# Autodesk Inventor assembly: Y_rail_Assembly_Rev3
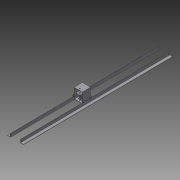
[picture p0: Inventor's stored thumbnail of the model, 180x180]
Saved by Autodesk Inventor 2015 (Build 190159000, 159)
## iProperties
Created: 2017-01-11
Part Number: Y_rail_Assembly_Rev3
Document SubType Name: Assembly
Designer: Guy
Mass: 1796.89 g
Surface Area: 4829.55 cm^2
Volume: 1200.62 cm^3
Density: 1.49664 g/cm^3
Author: Guy
## Documents named in this file (10)
- C:\Users\Guy\Documents\Fourth Year\Capstone\git\Capstone-Project\doc\CAD\LowLevel_Rev3\Y_rail_Assembly_Rev3.iam
- C:\Users\Guy\Documents\Fourth Year\Capstone\git\Capstone-Project\doc\CAD\LowLevel_Rev3\Y_Rail-SquareBar-Rev3.ipt
- C:\Users\Guy\Documents\Fourth Year\Capstone\git\Capstone-Project\doc\CAD\LowLevel_Rev3\XY_Wheel-SquareBar-Rev3.ipt
- C:\Users\Guy\Documents\Fourth Year\Capstone\git\Capstone-Project\doc\CAD\LowLevel_Rev3\EE_Base-SquareBar-Rev3.ipt
- C:\Users\Guy\Documents\Fourth Year\Capstone\git\Capstone-Project\doc\CAD\LowLevel_Rev3\Y_rail_Assembly_Rev3\Design Accelerator\Spur Gears1.iam
- C:\Users\Guy\Documents\Fourth Year\Capstone\git\Capstone-Project\doc\CAD\LowLevel_Rev3\Stepper_Motor_Holder-SquareBar-Rev3.ipt
- C:\Users\Guy\Documents\Fourth Year\Capstone\git\Capstone-Project\doc\CAD\Stepper Motor\NEMA 17-old\M1173041- NEMA 17.ipt
- C:\Users\Guy\Documents\Fourth Year\Capstone\git\Capstone-Project\doc\CAD\Nuts and Bolts\3-16in_1 1-4in_Bolt.ipt
- C:\Users\Guy\Documents\Fourth Year\Capstone\git\Capstone-Project\doc\CAD\Nuts and Bolts\3-16in_7-16in_washer(num8).ipt
- C:\Users\Guy\Documents\Fourth Year\Capstone\git\Capstone-Project\doc\CAD\Nuts and Bolts\3-16in_1-16in_nut(num2).ipt
## Components (34 placed, 9 different names)
1. Y_Rail-SquareBar-Rev3:1 — Tangent:1, Tangent:2, Mate:39, Mate:97, Mate:99
2. Y_Rail-SquareBar-Rev3:2 — Tangent:3, Tangent:4, Mate:12, Mate:97, Mate:99
3. XY_Wheel-SquareBar-Rev3:1 — Tangent:1, Mate:9, Flush:2, Mate:39, Mate:45, Mate:51
4. XY_Wheel-SquareBar-Rev3:2 — Tangent:4, Mate:9, Flush:4, Mate:15, Mate:71, Mate:84, Mate:92, Mate:95
5. XY_Wheel-SquareBar-Rev3:3 — Tangent:3, Mate:10, Mate:12, Flush:4, Mate:14, Mate:54, Mate:64, Mate:65
6. XY_Wheel-SquareBar-Rev3:4 — Tangent:2, Mate:10, Flush:2, Mate:13, Mate:73, Mate:79, Mate:80
7. Spur Gears:1 [sub-assembly] — Mate:17, Mate:36, Flush:5
8. EE_Base-SquareBar-Rev3:1 — Mate:13, Mate:14, Mate:15, Mate:17, Mate:37, Mate:38, Mate:53, Mate:55, Mate:63, Mate:68, Mate:69, Mate:71, Mate:72, Mate:74, Mate:85, Mate:88, Mate:98, Mate:100, Mate:101
9. M1173041- NEMA 17:1 — Mate:36, Flush:5, Mate:69, Mate:70, Mate:98
10. 3-16in_1 1-4in_Bolt:1 — Mate:37, Mate:38, Mate:44, Mate:46, Mate:48, Mate:49, Mate:52
11. 3-16in_7-16in_washer(num8):3 — Mate:44, Mate:45, Mate:47
12. 3-16in_1-16in_nut(num2):1 — Mate:46, Mate:47
13. 3-16in_7-16in_washer(num8):4 — Mate:48, Mate:50, Mate:51
14. 3-16in_1-16in_nut(num2):2 — Mate:49, Mate:50
15. 3-16in_1-16in_nut(num2):3 — Mate:52, Mate:53
16. 3-16in_1 1-4in_Bolt:2 — Mate:54, Mate:55, Mate:56, Mate:57, Mate:58, Mate:59, Mate:60
17. 3-16in_1-16in_nut(num2):4 — Mate:56, Mate:61
18. 3-16in_1-16in_nut(num2):5 — Mate:58, Mate:63
19. 3-16in_1-16in_nut(num2):6 — Mate:59, Mate:62
20. 3-16in_7-16in_washer(num8):5 — Mate:57, Mate:62, Mate:64
21. 3-16in_7-16in_washer(num8):6 — Mate:60, Mate:61, Mate:65
22. Stepper_Motor_Holder-SquareBar-Rev3:1 — Mate:68, Mate:70, Mate:100, Mate:101
23. 3-16in_1 1-4in_Bolt:3 — Mate:84, Mate:85, Mate:89, Mate:90, Mate:91, Mate:93, Mate:94
24. 3-16in_1 1-4in_Bolt:4 — Mate:72, Mate:73, Mate:75, Mate:77, Mate:78, Mate:82, Mate:83
25. 3-16in_1-16in_nut(num2):7 — Mate:86, Mate:91
26. 3-16in_1-16in_nut(num2):8 — Mate:87, Mate:94
27. 3-16in_1-16in_nut(num2):9 — Mate:88, Mate:89
28. 3-16in_1-16in_nut(num2):10 — Mate:76, Mate:78
29. 3-16in_1-16in_nut(num2):11 — Mate:81, Mate:82
30. 3-16in_1-16in_nut(num2):12 — Mate:74, Mate:75
31. 3-16in_7-16in_washer(num8):7 — Mate:80, Mate:81, Mate:83
32. 3-16in_7-16in_washer(num8):8 — Mate:87, Mate:93, Mate:95
33. 3-16in_7-16in_washer(num8):9 — Mate:76, Mate:77, Mate:79
34. 3-16in_7-16in_washer(num8):10 — Mate:86, Mate:90, Mate:92
## Relationships (73: Mate 66, Tangent 4, Flush 3)
- Tangent:1: Y_Rail-SquareBar-Rev3:1 ↔ XY_Wheel-SquareBar-Rev3:1
- Tangent:2: Y_Rail-SquareBar-Rev3:1 ↔ XY_Wheel-SquareBar-Rev3:4
- Tangent:3: Y_Rail-SquareBar-Rev3:2 ↔ XY_Wheel-SquareBar-Rev3:3
- Tangent:4: Y_Rail-SquareBar-Rev3:2 ↔ XY_Wheel-SquareBar-Rev3:2
- Mate:9: XY_Wheel-SquareBar-Rev3:1 ↔ XY_Wheel-SquareBar-Rev3:2
- Mate:10: XY_Wheel-SquareBar-Rev3:3 ↔ XY_Wheel-SquareBar-Rev3:4
- Flush:2: XY_Wheel-SquareBar-Rev3:1 ↔ XY_Wheel-SquareBar-Rev3:4
- Mate:12 (1.75 mm): Y_Rail-SquareBar-Rev3:2 ↔ XY_Wheel-SquareBar-Rev3:3
- Flush:4: XY_Wheel-SquareBar-Rev3:2 ↔ XY_Wheel-SquareBar-Rev3:3
- Mate:13: XY_Wheel-SquareBar-Rev3:4 ↔ EE_Base-SquareBar-Rev3:1
- Mate:14: XY_Wheel-SquareBar-Rev3:3 ↔ EE_Base-SquareBar-Rev3:1
- Mate:15: XY_Wheel-SquareBar-Rev3:2 ↔ EE_Base-SquareBar-Rev3:1
- Mate:17: Spur Gears:1 ↔ EE_Base-SquareBar-Rev3:1
- Mate:36: Spur Gears:1 ↔ M1173041- NEMA 17:1
- Flush:5 (-10 mm): Spur Gears:1 ↔ M1173041- NEMA 17:1
- Mate:37: EE_Base-SquareBar-Rev3:1 ↔ 3-16in_1 1-4in_Bolt:1
- Mate:38: EE_Base-SquareBar-Rev3:1 ↔ 3-16in_1 1-4in_Bolt:1
- Mate:39: Y_Rail-SquareBar-Rev3:1 ↔ XY_Wheel-SquareBar-Rev3:1
- Mate:44: 3-16in_1 1-4in_Bolt:1 ↔ 3-16in_7-16in_washer(num8):3
- Mate:45: XY_Wheel-SquareBar-Rev3:1 ↔ 3-16in_7-16in_washer(num8):3
- Mate:46: 3-16in_1 1-4in_Bolt:1 ↔ 3-16in_1-16in_nut(num2):1
- Mate:47: 3-16in_7-16in_washer(num8):3 ↔ 3-16in_1-16in_nut(num2):1
- Mate:48: 3-16in_1 1-4in_Bolt:1 ↔ 3-16in_7-16in_washer(num8):4
- Mate:49: 3-16in_1 1-4in_Bolt:1 ↔ 3-16in_1-16in_nut(num2):2
- Mate:50: 3-16in_7-16in_washer(num8):4 ↔ 3-16in_1-16in_nut(num2):2
- Mate:51: XY_Wheel-SquareBar-Rev3:1 ↔ 3-16in_7-16in_washer(num8):4
- Mate:52: 3-16in_1 1-4in_Bolt:1 ↔ 3-16in_1-16in_nut(num2):3
- Mate:53: EE_Base-SquareBar-Rev3:1 ↔ 3-16in_1-16in_nut(num2):3
- Mate:54: XY_Wheel-SquareBar-Rev3:3 ↔ 3-16in_1 1-4in_Bolt:2
- Mate:55: EE_Base-SquareBar-Rev3:1 ↔ 3-16in_1 1-4in_Bolt:2
- Mate:56: 3-16in_1 1-4in_Bolt:2 ↔ 3-16in_1-16in_nut(num2):4
- Mate:57: 3-16in_1 1-4in_Bolt:2 ↔ 3-16in_7-16in_washer(num8):5
- Mate:58: 3-16in_1 1-4in_Bolt:2 ↔ 3-16in_1-16in_nut(num2):5
- Mate:59: 3-16in_1 1-4in_Bolt:2 ↔ 3-16in_1-16in_nut(num2):6
- Mate:60: 3-16in_1 1-4in_Bolt:2 ↔ 3-16in_7-16in_washer(num8):6
- Mate:61: 3-16in_1-16in_nut(num2):4 ↔ 3-16in_7-16in_washer(num8):6
- Mate:62: 3-16in_1-16in_nut(num2):6 ↔ 3-16in_7-16in_washer(num8):5
- Mate:63: EE_Base-SquareBar-Rev3:1 ↔ 3-16in_1-16in_nut(num2):5
- Mate:64: XY_Wheel-SquareBar-Rev3:3 ↔ 3-16in_7-16in_washer(num8):5
- Mate:65: XY_Wheel-SquareBar-Rev3:3 ↔ 3-16in_7-16in_washer(num8):6
- Mate:68: EE_Base-SquareBar-Rev3:1 ↔ Stepper_Motor_Holder-SquareBar-Rev3:1
- Mate:69: EE_Base-SquareBar-Rev3:1 ↔ M1173041- NEMA 17:1
- Mate:70: M1173041- NEMA 17:1 ↔ Stepper_Motor_Holder-SquareBar-Rev3:1
- Mate:71 (5.625 mm): XY_Wheel-SquareBar-Rev3:2 ↔ EE_Base-SquareBar-Rev3:1
- Mate:72: EE_Base-SquareBar-Rev3:1 ↔ 3-16in_1 1-4in_Bolt:4
- Mate:73: XY_Wheel-SquareBar-Rev3:4 ↔ 3-16in_1 1-4in_Bolt:4
- Mate:74: EE_Base-SquareBar-Rev3:1 ↔ 3-16in_1-16in_nut(num2):12
- Mate:75: 3-16in_1 1-4in_Bolt:4 ↔ 3-16in_1-16in_nut(num2):12
- Mate:76: 3-16in_1-16in_nut(num2):10 ↔ 3-16in_7-16in_washer(num8):9
- Mate:77: 3-16in_1 1-4in_Bolt:4 ↔ 3-16in_7-16in_washer(num8):9
- Mate:78: 3-16in_1 1-4in_Bolt:4 ↔ 3-16in_1-16in_nut(num2):10
- Mate:79: XY_Wheel-SquareBar-Rev3:4 ↔ 3-16in_7-16in_washer(num8):9
- Mate:80: XY_Wheel-SquareBar-Rev3:4 ↔ 3-16in_7-16in_washer(num8):7
- Mate:81: 3-16in_1-16in_nut(num2):11 ↔ 3-16in_7-16in_washer(num8):7
- Mate:82: 3-16in_1 1-4in_Bolt:4 ↔ 3-16in_1-16in_nut(num2):11
- Mate:83: 3-16in_1 1-4in_Bolt:4 ↔ 3-16in_7-16in_washer(num8):7
- Mate:84: XY_Wheel-SquareBar-Rev3:2 ↔ 3-16in_1 1-4in_Bolt:3
- Mate:85: EE_Base-SquareBar-Rev3:1 ↔ 3-16in_1 1-4in_Bolt:3
- Mate:86: 3-16in_1-16in_nut(num2):7 ↔ 3-16in_7-16in_washer(num8):10
- Mate:87: 3-16in_1-16in_nut(num2):8 ↔ 3-16in_7-16in_washer(num8):8
- Mate:88: EE_Base-SquareBar-Rev3:1 ↔ 3-16in_1-16in_nut(num2):9
- Mate:89: 3-16in_1 1-4in_Bolt:3 ↔ 3-16in_1-16in_nut(num2):9
- Mate:90: 3-16in_1 1-4in_Bolt:3 ↔ 3-16in_7-16in_washer(num8):10
- Mate:91: 3-16in_1 1-4in_Bolt:3 ↔ 3-16in_1-16in_nut(num2):7
- Mate:92: XY_Wheel-SquareBar-Rev3:2 ↔ 3-16in_7-16in_washer(num8):10
- Mate:93: 3-16in_1 1-4in_Bolt:3 ↔ 3-16in_7-16in_washer(num8):8
- Mate:94: 3-16in_1 1-4in_Bolt:3 ↔ 3-16in_1-16in_nut(num2):8
- Mate:95: XY_Wheel-SquareBar-Rev3:2 ↔ 3-16in_7-16in_washer(num8):8
- Mate:97: Y_Rail-SquareBar-Rev3:1 ↔ Y_Rail-SquareBar-Rev3:2
- Mate:98 (45.4267 mm): EE_Base-SquareBar-Rev3:1 ↔ M1173041- NEMA 17:1
- Mate:99 (95 mm): Y_Rail-SquareBar-Rev3:1 ↔ Y_Rail-SquareBar-Rev3:2
- Mate:100: EE_Base-SquareBar-Rev3:1 ↔ Stepper_Motor_Holder-SquareBar-Rev3:1
- Mate:101: EE_Base-SquareBar-Rev3:1 ↔ Stepper_Motor_Holder-SquareBar-Rev3:1
